# Autodesk Inventor assembly: Assembly1
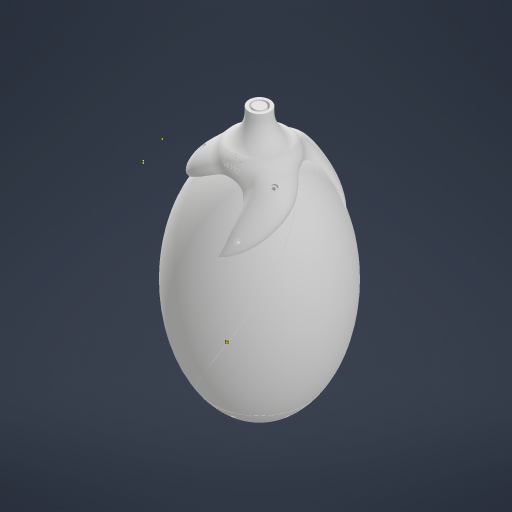
[picture p0: Inventor's stored thumbnail of the model, 512x512]
Saved by Autodesk Inventor 2023 (Build 270158000, 158)
## iProperties
Created: 2022-06-17
Part Number: Assembly1
Document SubType Name: Assembly
Designer: bananenbrot
Author: bananenbrot
## Documents named in this file (9)
- D:\fusion-zauberstab\inventor\Assembly1.iam
- D:\fusion-zauberstab\inventor\vase_v2._tom.ipt
- D:\fusion-zauberstab\inventor\Spant.ipt
- D:\fusion-zauberstab\inventor\top_centering_ring.ipt
- D:\fusion-zauberstab\inventor\lower_centering_ring.ipt
- D:\fusion-zauberstab\inventor\Spant2.ipt
- D:\fusion-zauberstab\inventor\deckel.ipt
- D:\fusion-zauberstab\inventor\boden.ipt
- D:\fusion-zauberstab\inventor\aufhaengung.ipt
## Components (12 placed, 8 different names)
1. vase_v2._tom:1 — Mate:1, Mate:2, Flush:2, Flush:3, Flush:4, Flush:5, Flush:7, Mate:3, Angle:1, Flush:8, Flush:9, Mate:5, Flush:10, Mate:7, Flush:11, Flush:13, Mate:8
2. top_centering_ring:1 — Flush:4, Flush:5, Mate:4
3. lower_centering_ring:1 — Flush:7, Mate:6
4. deckel:1 — Mate:4, Mate:5, Flush:10
5. boden:1 — Mate:6, Mate:7, Flush:11, Flush:14, Mate:9
6. aufhaengung:1 — Flush:12, Flush:13, Flush:14, Mate:8, Mate:9
7. Spant:1 — Flush:1, Flush:3
8. Spant:2
9. Spant:3
10. Spant2:1 — Flush:8, Flush:9
11. Spant2:2
12. Spant2:3
## Component patterns: (3 elements, first: Spant:1), (3 elements, first: Spant2:1)
## Relationships (23: Flush 13, Mate 9, Angle 1)
- Mate:1: vase_v2._tom:1
- Mate:2: vase_v2._tom:1
- Flush:1: Spant:1
- Flush:2: vase_v2._tom:1
- Flush:3: vase_v2._tom:1 ↔ Spant:1
- Flush:4: vase_v2._tom:1 ↔ top_centering_ring:1
- Flush:5: vase_v2._tom:1 ↔ top_centering_ring:1
- Flush:7: vase_v2._tom:1 ↔ lower_centering_ring:1
- Mate:3: vase_v2._tom:1
- Angle:1 (45 deg): vase_v2._tom:1
- Flush:8: vase_v2._tom:1 ↔ Spant2:1
- Flush:9: vase_v2._tom:1 ↔ Spant2:1
- Mate:4: top_centering_ring:1 ↔ deckel:1
- Mate:5: vase_v2._tom:1 ↔ deckel:1
- Flush:10: vase_v2._tom:1 ↔ deckel:1
- Mate:6: lower_centering_ring:1 ↔ boden:1
- Mate:7: vase_v2._tom:1 ↔ boden:1
- Flush:11: vase_v2._tom:1 ↔ boden:1
- Flush:12: aufhaengung:1
- Flush:13 (3.9878 mm): vase_v2._tom:1 ↔ aufhaengung:1
- Flush:14 (3.9878 mm): boden:1 ↔ aufhaengung:1
- Mate:8: vase_v2._tom:1 ↔ aufhaengung:1
- Mate:9: boden:1 ↔ aufhaengung:1
